# Autodesk Inventor assembly: wheel5
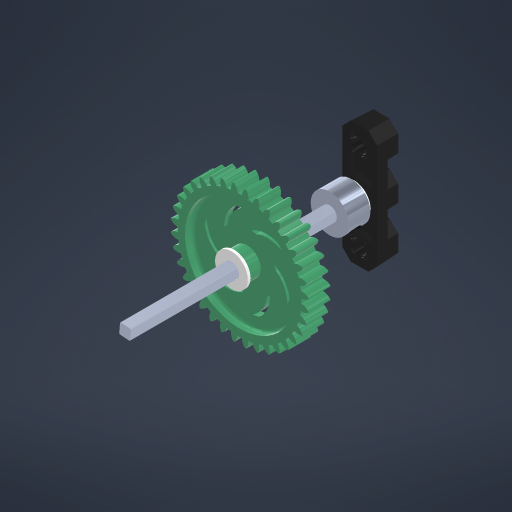
[picture p0: Inventor's stored thumbnail of the model, 512x512]
Saved by Autodesk Inventor 2024 (Build 280153000, 153)
## iProperties
Created: 2023-08-09
Part Number: wheel5
Document SubType Name: Assembly
Designer: macbook
Author: macbook
## Documents named in this file (15)
- \\Mac\Home\Desktop\code\7899V-VRC-OVER-UNDER\Cad\VEX-CAD-Inventor-1.4.0\Assembly\v0.2\wheel5.iam
- \\Mac\Home\Desktop\code\7899V-VRC-OVER-UNDER\Cad\VEX-CAD-Inventor-1.4.0\Motion\Gears\LS 36T Gear.ipt
- \\Mac\Home\Desktop\code\7899V-VRC-OVER-UNDER\Cad\VEX-CAD-Inventor-1.4.0\Motion\Shaft LS\Bearing Flat.ipt
- \\Mac\Home\Desktop\code\7899V-VRC-OVER-UNDER\Cad\VEX-CAD-Inventor-1.4.0\Motion\Shaft LS\Shaft LS\Shaft LS 3.0.ipt
- \\Mac\Home\Desktop\code\7899V-VRC-OVER-UNDER\Cad\VEX-CAD-Inventor-1.4.0\Motion\Shaft LS\Shaft LS.ipt
- \\Mac\Home\Desktop\code\7899V-VRC-OVER-UNDER\Cad\VEX-CAD-Inventor-1.4.0\Motion\Shaft LS\Shaft Collar Metal\Shaft Collar Set Screw.iam
- \\Mac\Home\Desktop\code\7899V-VRC-OVER-UNDER\Cad\VEX-CAD-Inventor-1.4.0\Motion\Shaft LS\Shaft Collar Metal.iam
- \\Mac\Home\Desktop\code\7899V-VRC-OVER-UNDER\Cad\VEX-CAD-Inventor-1.4.0\Motion\Spacers\Washer Teflon\TWasher .375 OD x .03125.ipt
- \\Mac\Home\Desktop\code\7899V-VRC-OVER-UNDER\Cad\VEX-CAD-Inventor-1.4.0\Motion\Spacers\Washer Teflon.ipt
- \\Mac\Home\Desktop\code\7899V-VRC-OVER-UNDER\Cad\VEX-CAD-Inventor-1.4.0\Motion\Shaft HS\HS Bearing Flat.ipt
- \\Mac\Home\Desktop\code\7899V-VRC-OVER-UNDER\Cad\VEX-CAD-Inventor-1.4.0\Structure\Standoff.ipt
- \\Mac\Home\Desktop\code\7899V-VRC-OVER-UNDER\Cad\VEX-CAD-Inventor-1.4.0\Motion\Gears\HS Gear\HS 36T Gear, Circle.iam
- \\Mac\Home\Desktop\code\7899V-VRC-OVER-UNDER\Cad\VEX-CAD-Inventor-1.4.0\Motion\Gears\HS Gear.iam
- \\Mac\Home\Desktop\code\7899V-VRC-OVER-UNDER\Cad\VEX-CAD-Inventor-1.4.0\Structure\Standoff\Standoff 2.00.ipt
- \\Mac\Home\Desktop\code\7899V-VRC-OVER-UNDER\Cad\VEX-CAD-Inventor-1.4.0\Motion\Pneumatics\Double Acting Piston.iam
## Components (14 placed, 9 different names)
1. LS 36T Gear:1
2. Bearing Flat:1
3. Shaft LS 3.0:1
4. Shaft Collar Set Screw:1 [sub-assembly]
5. Shaft Collar Set Screw:2 [sub-assembly]
6. TWasher .375 OD x .03125:1
7. TWasher .375 OD x .03125:2
8. Standoff 2.00:1
9. HS 36T Gear, Circle:1 [sub-assembly] — Insert:10, Insert:11, Insert:12, Insert:13
10. LS 36T Gear:2
11. LS 36T Gear:3
12. HS Bearing Flat:3 — Insert:10, Insert:11
13. HS Bearing Flat:4 — Insert:12, Insert:13
14. Double Acting Piston:1 [sub-assembly]
## Relationships (11: Insert 8, CylindricalJoint 2, Flush 1)
- [Insert]: LS 36T Gear:1 ↔ TWasher .375 OD x .03125:1
- [Insert]: LS 36T Gear:1 ↔ Shaft Collar Set Screw:2
- [CylindricalJoint]: Shaft LS 3.0:1 ↔ Shaft Collar Set Screw:2
- [Flush] (1.5875 mm): Bearing Flat:1 ↔ Shaft LS 3.0:1
- [CylindricalJoint]: Bearing Flat:1 ↔ Shaft LS 3.0:1
- [Insert]: Shaft Collar Set Screw:1 ↔ TWasher .375 OD x .03125:2
- [Insert] (1.5875 mm): Bearing Flat:1 ↔ TWasher .375 OD x .03125:2
- Insert:10: HS 36T Gear, Circle:1 ↔ HS Bearing Flat:3
- Insert:11: HS 36T Gear, Circle:1 ↔ HS Bearing Flat:3
- Insert:12: HS 36T Gear, Circle:1 ↔ HS Bearing Flat:4
- Insert:13: HS 36T Gear, Circle:1 ↔ HS Bearing Flat:4
